# Autodesk Inventor assembly: czlon 1 i 2
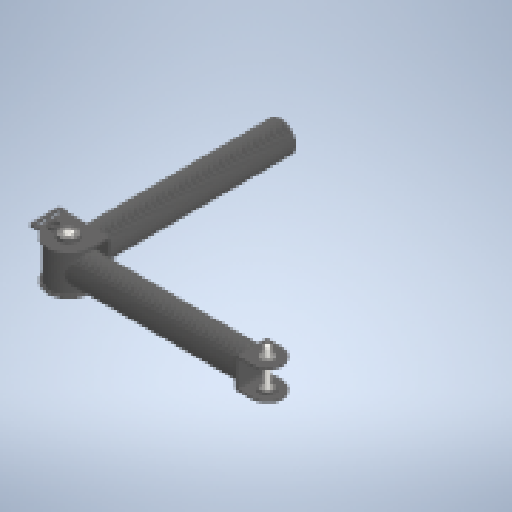
[picture p0: Inventor's stored thumbnail of the model, 512x512]
Saved by Autodesk Inventor 2023 (Build 270158000, 158)
## iProperties
Created: 2023-04-09
Part Number: czlon 1 i 2
Document SubType Name: Assembly
Designer: Wiktor
Mass: 5411.46 g
Surface Area: 10600.9 cm^2
Volume: 2825.09 cm^3
Density: 1.9155 g/cm^3
Author: Wiktor
## Documents named in this file (9)
- C:\Users\krzys\Documents\GitHub\Manipulator-Inventor\czlon 1 i 2.iam
- C:\Users\krzys\Documents\GitHub\Manipulator-Inventor\czlon i przekladnia.iam
- C:\Users\krzys\Documents\GitHub\Manipulator-Inventor\Wał1.ipt
- C:\Users\krzys\Documents\GitHub\Manipulator-Inventor\czlon 1 i 2\Design Accelerator\Połączenie wpustowe1.iam
- C:\Users\krzys\Documents\GitHub\Manipulator-Inventor\czlon 2.ipt
- C:\Users\krzys\Documents\GitHub\Manipulator-Inventor\czlon 1 i 2\Design Accelerator\Łożysko2.iam
- C:\Users\krzys\Documents\GitHub\Manipulator-Inventor\Wał3.ipt
- C:\Users\krzys\Documents\GitHub\Manipulator-Inventor\czlon 1 i 2\Design Accelerator\Łożysko3.iam
- C:\Users\krzys\Documents\GitHub\Manipulator-Inventor\czlon 1 i 2\Design Accelerator\Łożysko4.iam
## Components (9 placed, 5 different names)
1. czlon i przekladnia:1 [sub-assembly] — Równoległe:1, Wstawiające:5, Wstawiające:6
2. Wał:1 — Zestawiające:10, Wstawiające:4
3. Połączenie wpustowe:1 [sub-assembly]
4. czlon 2:1 — Zestawiające:10, Równoległe:1, Wstawiające:2, Wstawiające:3
5. Łożysko:4 [sub-assembly] — Wstawiające:3, Zestawiające:11, Równoległe:2, Kątowe:2
6. Łożysko:5 [sub-assembly] — Wstawiające:2
7. Wał:1 — Zestawiające:11, Równoległe:2, Kątowe:2
8. Łożysko:6 [sub-assembly] — Wstawiające:4, Wstawiające:6
9. Łożysko:7 [sub-assembly] — Wstawiające:5
## Relationships (10: Insert 5, Mate 2, Flush 2, Angle 1)
- Zestawiające:10 [Mate]: Wał:1 ↔ czlon 2:1
- Równoległe:1 [Flush]: czlon i przekladnia:1 ↔ czlon 2:1
- Wstawiające:2 [Insert]: czlon 2:1 ↔ Łożysko:5
- Wstawiające:3 [Insert]: czlon 2:1 ↔ Łożysko:4
- Zestawiające:11 [Mate]: Łożysko:4 ↔ Wał:1
- Równoległe:2 [Flush]: Łożysko:4 ↔ Wał:1
- Kątowe:2 [Angle] (0 deg): Łożysko:4 ↔ Wał:1
- Wstawiające:4 [Insert] (-1 mm): Wał:1 ↔ Łożysko:6
- Wstawiające:5 [Insert] (-1 mm): czlon i przekladnia:1 ↔ Łożysko:7
- Wstawiające:6 [Insert]: czlon i przekladnia:1 ↔ Łożysko:6
